# Autodesk Inventor assembly: motor-mount
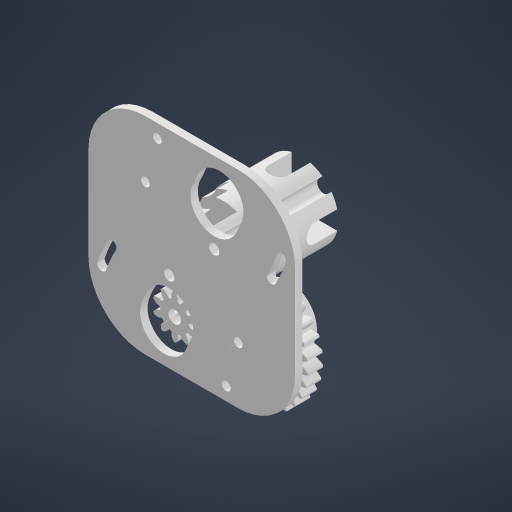
[picture p0: Inventor's stored thumbnail of the model, 512x512]
Saved by Autodesk Inventor 2024 (Build 280153000, 153)
## iProperties
Created: 2024-05-16
Part Number: motor-mount
Document SubType Name: Assembly
Designer: loren
elephant_prevention_radius: 0,300 mm
Author: loren
## Documents named in this file (7)
- C:\Users\lokies\Nextcloud\projects\motorized-mounts\mechanical\pancake-geared\pancake-geared.iam
- C:\Users\lokies\Nextcloud\projects\motorized-mounts\mechanical\pancake-geared\mount-plate.ipt
- C:\Users\lokies\Nextcloud\projects\motorized-mounts\mechanical\pancake-geared\gear.ipt
- C:\Users\lokies\Nextcloud\projects\motorized-mounts\mechanical\pancake-geared\screw-grip.ipt
- C:\Users\lokies\Nextcloud\projects\motorized-mounts\mechanical\pancake-geared\mount-stem.ipt
- C:\Users\lokies\Nextcloud\projects\motorized-mounts\mechanical\pancake-geared\pinion.ipt
- C:\Users\lokies\Nextcloud\projects\motorized-mounts\mechanical\pancake-geared\params.xlsx
## Components (5 placed, 5 different names)
1. mount-plate:1 — Mate:1, Mate:2, Mate:6, Mate:8, Flush:3, Mate:10
2. gear:1 — Mate:1, Mate:2, Mate:3, Flush:1, Flush:2, Mate:7
3. screw-grip:1 — Mate:3, Flush:1, Flush:2
4. pinion:1 — Mate:6, Mate:7, Mate:8
5. mount-stem:1 — Flush:3, Mate:9, Mate:10
## Relationships (11: Mate 8, Flush 3)
- Mate:1: mount-plate:1 ↔ gear:1
- Mate:2 (1 mm): mount-plate:1 ↔ gear:1
- Mate:3: gear:1 ↔ screw-grip:1
- Flush:1: gear:1 ↔ screw-grip:1
- Flush:2: gear:1 ↔ screw-grip:1
- Mate:6 (0.5 mm): mount-plate:1 ↔ pinion:1
- Mate:7 (25 mm): gear:1 ↔ pinion:1
- Mate:8 (21.925 mm): mount-plate:1 ↔ pinion:1
- Flush:3: mount-plate:1 ↔ mount-stem:1
- Mate:9: mount-stem:1
- Mate:10: mount-plate:1 ↔ mount-stem:1
## Named parameters: thumbscrew_dia = 15.8 mm, helix_length = 3.5 mm, helix_width = 2 mm, helix_fillet = 0.3 mm, helix_teeth = 8, helix_inner_dia = 19 mm, helix_outer_dia = 23 mm, elephant_prevention_radius = 0.3 mm, gear_center_distance = 25 mm, stepper_screw_dist = 43.85 mm, stepper_axis_offset = 0 mm, stepper_axis_clearance = 16.5 mm, mount_screw_ortho_dist = 31 mm, stepper_dia = 36.3 mm, sheet_thick = 2.5 mm, helix_winding_factor = 1.2
